# Autodesk Inventor assembly: tetrix_739197_2012
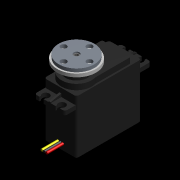
[picture p0: Inventor's stored thumbnail of the model, 180x180]
Saved by Autodesk Inventor 2015 SP1 (Build 190203100, 203)
## iProperties
Created: 2015-01-25
Part Number: tetrix_739197_2012
Document SubType Name: Assembly
Designer: rihoobler
Author: Kyle
Title: C:\Users\Kyle\Documents\Tetrix_Kit_FTC\tetrix_739197_2012.stp
Creation Date: 2013-08-31
Sending System: Autodesk Inventor 2014
Preprocessor: ST-DEVELOPER v15.2
Author: rihoobler
## Documents named in this file (5)
- C:\Users\datenney\Documents\GitHub\CAD\SerenityMk.2\Imported Components\tetrix_739197_2012\tetrix_739197_2012.iam
- C:\Users\datenney\Documents\GitHub\CAD\SerenityMk.2\Imported Components\tetrix_739197_2012\TETRIX_739197_SERVO_2012.ipt
- C:\Users\datenney\Documents\GitHub\CAD\SerenityMk.2\Imported Components\tetrix_739197_2012\TETRIX_739197_METAL_HORN_2012.ipt
- C:\Users\datenney\Documents\GitHub\CAD\SerenityMk.2\Imported Components\tetrix_739197_2012\TETRIX_739197_SCREW_2012.ipt
- C:\Users\datenney\Documents\GitHub\CAD\SerenityMk.2\Imported Components\tetrix_739197_2012\TETRIX_739197_PLASTIC_HORN_2012.ipt
## Components (4 placed, 4 different names)
1. TETRIX_739197_SERVO_2012:1 — Mate:2, Mate:6
2. TETRIX_739197_METAL_HORN_2012:1 — Mate:1, Mate:3, Mate:5, Rotation:2
3. TETRIX_739197_SCREW_2012:1 — Mate:2, Mate:3, Mate:4
4. TETRIX_739197_PLASTIC_HORN_2012:1 — Mate:1, Mate:4, Mate:5, Mate:6, Rotation:2
## Relationships (7: Mate 6, RelateRotation 1)
- Mate:1: TETRIX_739197_METAL_HORN_2012:1 ↔ TETRIX_739197_PLASTIC_HORN_2012:1
- Mate:2: TETRIX_739197_SERVO_2012:1 ↔ TETRIX_739197_SCREW_2012:1
- Mate:3: TETRIX_739197_METAL_HORN_2012:1 ↔ TETRIX_739197_SCREW_2012:1
- Mate:4: TETRIX_739197_SCREW_2012:1 ↔ TETRIX_739197_PLASTIC_HORN_2012:1
- Mate:5: TETRIX_739197_METAL_HORN_2012:1 ↔ TETRIX_739197_PLASTIC_HORN_2012:1
- Mate:6: TETRIX_739197_SERVO_2012:1 ↔ TETRIX_739197_PLASTIC_HORN_2012:1
- Rotation:2 [RelateRotation] (1.091 ul): TETRIX_739197_METAL_HORN_2012:1 ↔ TETRIX_739197_PLASTIC_HORN_2012:1
